# Autodesk Inventor assembly: Omni Wheel Assembly
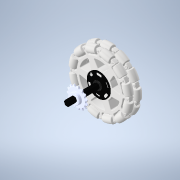
[picture p0: Inventor's stored thumbnail of the model, 180x180]
Saved by Autodesk Inventor 2020 (Build 240168000, 168)
## iProperties
Created: 2020-01-25
Part Number: Omni Wheel Assembly
Document SubType Name: Assembly
Designer: aidan
Author: aidan
## Documents named in this file (6)
- C:\Users\aidan\Desktop\T3 Robotics\CAD\Omni Wheel Assembly.iam
- C:\Users\aidan\Desktop\T3 Robotics\CAD\0.5in Hex Hub.ipt
- C:\Users\aidan\Desktop\T3 Robotics\CAD\STEP Files\6_Omni-Directional_Wheel_217-2585.ipt
- C:\Users\aidan\Desktop\T3 Robotics\CAD\5.5 thundershaft.ipt
- C:\Users\aidan\Desktop\T3 Robotics\CAD\Generic and Stock\Hex Spacer STOCK.ipt
- C:\Users\aidan\Desktop\T3 Robotics\CAD\Generic and Stock\15T Sprocket.ipt
## Components (7 placed, 5 different names)
1. 0.5in Hex Hub:1 — Mate:1, Mate:2, Mate:3, Flush:1, Mate:7, Mate:8
2. 0.5in Hex Hub:2 — Mate:4, Mate:5, Mate:6, Mate:11
3. 6_Omni-Directional_Wheel_217-2585:1 — Mate:1, Mate:2, Mate:3, Mate:4, Mate:5, Mate:6
4. 5.5 thundershaft:1 — Flush:1, Mate:7, Mate:8, Mate:9, Mate:10, Mate:13, Mate:14, Mate:16, Mate:17, Mate:18, Mate:19, Angle:1
5. Hex Spacer STOCK:1 — Mate:12, Mate:13, Mate:14, Mate:15
6. Hex Spacer STOCK:2 — Mate:9, Mate:10, Mate:11, Mate:12
7. 15T Sprocket:1 — Mate:15, Mate:16, Mate:17
## Relationships (23: Mate 21, Flush 1, Angle 1)
- Mate:1: 0.5in Hex Hub:1 ↔ 6_Omni-Directional_Wheel_217-2585:1
- Mate:2: 0.5in Hex Hub:1 ↔ 6_Omni-Directional_Wheel_217-2585:1
- Mate:3: 0.5in Hex Hub:1 ↔ 6_Omni-Directional_Wheel_217-2585:1
- Mate:4: 0.5in Hex Hub:2 ↔ 6_Omni-Directional_Wheel_217-2585:1
- Mate:5: 0.5in Hex Hub:2 ↔ 6_Omni-Directional_Wheel_217-2585:1
- Mate:6: 0.5in Hex Hub:2 ↔ 6_Omni-Directional_Wheel_217-2585:1
- Flush:1: 0.5in Hex Hub:1 ↔ 5.5 thundershaft:1
- Mate:7: 0.5in Hex Hub:1 ↔ 5.5 thundershaft:1
- Mate:8: 0.5in Hex Hub:1 ↔ 5.5 thundershaft:1
- Mate:9: 5.5 thundershaft:1 ↔ Hex Spacer STOCK:2
- Mate:10: 5.5 thundershaft:1 ↔ Hex Spacer STOCK:2
- Mate:11: 0.5in Hex Hub:2 ↔ Hex Spacer STOCK:2
- Mate:12 (41.91 mm): Hex Spacer STOCK:1 ↔ Hex Spacer STOCK:2
- Mate:13: 5.5 thundershaft:1 ↔ Hex Spacer STOCK:1
- Mate:14: 5.5 thundershaft:1 ↔ Hex Spacer STOCK:1
- Mate:15: Hex Spacer STOCK:1 ↔ 15T Sprocket:1
- Mate:16: 5.5 thundershaft:1 ↔ 15T Sprocket:1
- Mate:17: 5.5 thundershaft:1 ↔ 15T Sprocket:1
- Mate:18: 5.5 thundershaft:1
- Mate:19: 5.5 thundershaft:1
- Mate:20
- Mate:21
- Angle:1 (0 deg): 5.5 thundershaft:1
